# Autodesk Inventor assembly: Tetrix_739901
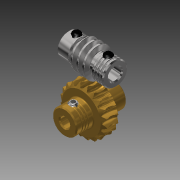
[picture p0: Inventor's stored thumbnail of the model, 180x180]
Saved by Autodesk Inventor 2015 SP1 (Build 190203100, 203)
## iProperties
Created: 2014-11-25
Part Number: Tetrix_739901
Document SubType Name: Assembly
Designer: Philip
Author: Philip
## Documents named in this file (5)
- D:\Data Folder\FTC 2015\KOP\Tetrix\Tetrix_739901.iam
- D:\Data Folder\FTC 2015\KOP\Tetrix\Tetrix_739901_Gear.ipt
- D:\Data Folder\FTC 2015\KOP\Tetrix\Tetrix_739901_Screw1.ipt
- D:\Data Folder\FTC 2015\KOP\Tetrix\Tetrix_739901_Worm.ipt
- D:\Data Folder\FTC 2015\KOP\Tetrix\Tetrix_739901_Screw2.ipt
## Components (6 placed, 4 different names)
1. Tetrix_739901_Gear:1 — Mate:1, Mate:2
2. Tetrix_739901_Screw1:1 — Mate:1
3. Tetrix_739901_Screw1:2 — Mate:2
4. Tetrix_739901_Worm:1 — Mate:3, Mate:4, Flush:2
5. Tetrix_739901_Screw2:1 — Mate:3, Flush:1, Flush:2
6. Tetrix_739901_Screw2:2 — Mate:4, Flush:1
## Relationships (6: Mate 4, Flush 2)
- Mate:1: Tetrix_739901_Gear:1 ↔ Tetrix_739901_Screw1:1
- Mate:2: Tetrix_739901_Gear:1 ↔ Tetrix_739901_Screw1:2
- Mate:3: Tetrix_739901_Worm:1 ↔ Tetrix_739901_Screw2:1
- Mate:4: Tetrix_739901_Worm:1 ↔ Tetrix_739901_Screw2:2
- Flush:1: Tetrix_739901_Screw2:1 ↔ Tetrix_739901_Screw2:2
- Flush:2 (-24 mm): Tetrix_739901_Worm:1 ↔ Tetrix_739901_Screw2:1
